# Autodesk Inventor assembly: hph_002
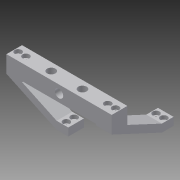
[picture p0: Inventor's stored thumbnail of the model, 180x180]
Saved by Autodesk Inventor 2014 (Build 180170000, 170)
## iProperties
Created: 2014-03-27
Part Number: hph_002
Document SubType Name: Assembly
Designer: stephenholtz
Author: stephenholtz
## Documents named in this file (3)
- C:\Users\stephenholtz\Dropbox\grad_school_docs\sabatini_lab_rotation\headpost_design\hph_002.iam
- C:\Users\stephenholtz\Dropbox\grad_school_docs\sabatini_lab_rotation\headpost_design\hph_C_001.ipt
- C:\Users\stephenholtz\Dropbox\grad_school_docs\sabatini_lab_rotation\headpost_design\hph_B_001.ipt
## Components (3 placed, 2 different names)
1. hph_C_001:1 — Rigid:1, Rigid:2
2. hph_B_001:1 — Rigid:1
3. hph_B_001:2 — Rigid:2
## Relationships (2: WeldJoint 2)
- Rigid:1 [WeldJoint]: hph_C_001:1 ↔ hph_B_001:1
- Rigid:2 [WeldJoint]: hph_C_001:1 ↔ hph_B_001:2
